# Autodesk Inventor assembly: Filament Motion Sensor Left
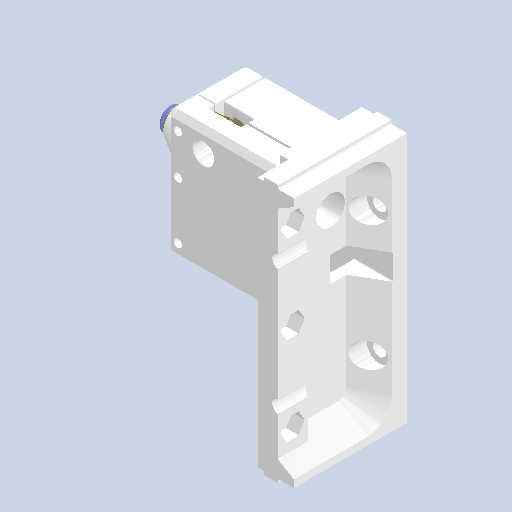
[picture p0: Inventor's stored thumbnail of the model, 512x512]
Saved by Autodesk Inventor 2024 (Build 280153000, 153)
## iProperties
Created: 2024-08-17
Part Number: Filament Motion Sensor Left
Document SubType Name: Assembly
Designer: Ishaan
Author: Ishaan
## Documents named in this file (7)
- E:\Projects\Axiom--IDEX-3D-Printer\CAD\05 - Filament Path\Filament Motion Sensor Left.iam
- E:\Projects\Axiom--IDEX-3D-Printer\CAD\05 - Filament Path\Filament Motion Sensor Left.ipt
- E:\Projects\Axiom--IDEX-3D-Printer\CAD\00 - COTS Components\ECAS Bowden Fitting\ECAS v1 (8).iam
- E:\Projects\Axiom--IDEX-3D-Printer\CAD\00 - COTS Components\ERCF Binky\ERCF Binky - 3D v1_1.iam
- E:\Projects\Axiom--IDEX-3D-Printer\CAD\00 - COTS Components\ERCF BondTech Drive Gear\BondTech Direct Drive Gear v1 (without screwset).iam
- E:\Projects\Axiom--IDEX-3D-Printer\CAD\05 - Filament Path\Filament Sensor Slotted Disk.ipt
- E:\Projects\Axiom--IDEX-3D-Printer\CAD\00 - COTS Components\V623ZZ.ipt
## Components (7 placed, 6 different names)
1. Filament Motion Sensor Left:1 — Insert:1, Insert:2, Insert:3, Angle:1, Mate:1, Mate:2, Mate:6, Mate:7
2. ECAS v1 (8):1 [sub-assembly] — Insert:1
3. ECAS v1 (8):2 [sub-assembly] — Insert:2
4. ERCF Binky - 3D v1_1:1 [sub-assembly] — Insert:3, Angle:1
5. BondTech Direct Drive Gear v1 (without screwset):1 [sub-assembly] — Mate:1, Mate:2, Insert:4
6. Filament Sensor Slotted Disk:1 — Insert:4
7. V623ZZ:1 — Mate:6, Mate:7
## Relationships (9: Insert 4, Mate 4, Angle 1)
- Insert:1: Filament Motion Sensor Left:1 ↔ ECAS v1 (8):1
- Insert:2: Filament Motion Sensor Left:1 ↔ ECAS v1 (8):2
- Insert:3: Filament Motion Sensor Left:1 ↔ ERCF Binky - 3D v1_1:1
- Angle:1 (180 deg): Filament Motion Sensor Left:1 ↔ ERCF Binky - 3D v1_1:1
- Mate:1: Filament Motion Sensor Left:1 ↔ BondTech Direct Drive Gear v1 (without screwset):1
- Mate:2: Filament Motion Sensor Left:1 ↔ BondTech Direct Drive Gear v1 (without screwset):1
- Insert:4 (0.1 mm): BondTech Direct Drive Gear v1 (without screwset):1 ↔ Filament Sensor Slotted Disk:1
- Mate:6: Filament Motion Sensor Left:1 ↔ V623ZZ:1
- Mate:7: Filament Motion Sensor Left:1 ↔ V623ZZ:1
